# Autodesk Inventor assembly: Aufhängung_Koppeltest
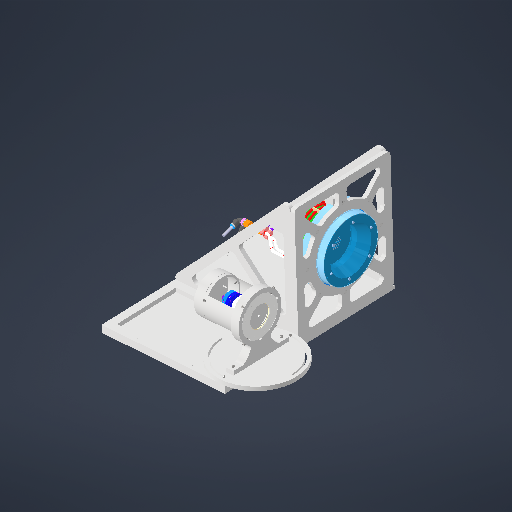
[picture p0: Inventor's stored thumbnail of the model, 512x512]
Saved by Autodesk Inventor 2027 (Build 310192060, 192F)
## iProperties
Created: 2026-07-21
Part Number: Aufhängung_Koppeltest
Document SubType Name: Assembly
Designer: kw
Author: kw
## Documents named in this file (13)
- C:\Users\kw\Documents\ABEP_Koppeltest\Koppeltest_Halterung - Kopie\Aufhängung_Koppeltest.iam
- C:\Users\kw\Documents\ABEP_Koppeltest\Koppeltest_Halterung - Kopie\Aufhängung_Seitenteil.ipt
- C:\Users\kw\Documents\ABEP_Koppeltest\Koppeltest_Halterung - Kopie\Halterung_Teflonplatte.ipt
- C:\Users\kw\Documents\ABEP_Koppeltest\Koppeltest_Halterung - Kopie\Pratze_ISO-K160.ipt
- C:\Users\kw\Documents\ABEP_Koppeltest\19K_001_010_00_A_RIM_10_2019_EFRE_3D_2024_0228\19K_001_010_00_A_RIM_10_2019_EFRE_3D_2024_0228.ipt
- C:\Users\kw\Documents\ABEP_Koppeltest\Koppeltest_Halterung - Kopie\Aufhängung_Front_Koppeltest.ipt
- C:\Users\kw\Documents\ABEP_Koppeltest\Koppeltest_Halterung - Kopie\Aufhängung_Front_RFG_Koppeltest.ipt
- C:\Users\kw\Documents\ABEP_Koppeltest\Koppeltest_Halterung - Kopie\Aufhängung_Drehscheibe.ipt
- C:\Users\kw\Documents\ABEP_Koppeltest\Koppeltest_Halterung - Kopie\Aufhängung_Seitenteil_Koppeltest_außen.ipt
- C:\Users\kw\Documents\ABEP_Koppeltest\RF-Neutralisator\RFN-Setup_Vol3.iam
- C:\Users\kw\OneDrive\Documents\Inventor\Content Center Files\R2027\en-US\ISO 4762(2)\ISO 4762 - M3 x 12ISO.ipt
- C:\Users\kw\OneDrive\Documents\Inventor\Content Center Files\R2027\en-US\ISO 4762(2)\ISO 4762 - M3 x 16ISO.ipt
- C:\Users\kw\OneDrive\Documents\Inventor\Content Center Files\R2027\en-US\ISO 4762(2)\ISO 4762 - M3 x 20ISO.ipt
## Components (18 placed, 12 different names)
1. Aufhängung_Seitenteil:1 — Flush:2, Flush:3, Mate:17, Mate:37, Mate:38
2. Pratze_ISO-K160:4 — Mate:5, Flush:7, Mate:28
3. 19K_001_010_00_A_RIM_10_2019_EFRE_3D_2024_0228:1 — Mate:3, Mate:4, Mate:28
4. Aufhängung_Front_Koppeltest:1 — Mate:2, Flush:5, Mate:3, Mate:4, Mate:5, Flush:7, Flush:13
5. Halterung_Teflonplatte:1 — Flush:2, Flush:3, Mate:2, Flush:5, Mate:17, Flush:13, Mate:37, Mate:38, Mate:39, Flush:17, Flush:18, Mate:40, Flush:19, Mate:41, Mate:42, Mate:43, Mate:44
6. Aufhängung_Front_RFG_Koppeltest:1 — Mate:16, Mate:32, Mate:33, Mate:34, Mate:35, Flush:16, Insert:1, Insert:2
7. Aufhängung_Drehscheibe:1 — Mate:16, Mate:32, Mate:33, Mate:47, Mate:48, Mate:49, Mate:50, Mate:51
8. Aufhängung_Seitenteil_Koppeltest_außen:1 — Mate:40, Flush:19, Mate:41, Mate:42, Mate:43, Mate:44, Mate:47, Mate:52, Mate:53
9. RFN-Setup_Vol3:1 [sub-assembly] — Mate:34, Mate:36, Flush:16
10. Aufhängung_Seitenteil:2 — Mate:39, Flush:17, Flush:18
11. ISO 4762 M3 x 16:1 — Mate:48, Mate:51, Mate:53
12. ISO 4762 M3 x 16:2 — Mate:49, Mate:50, Mate:52
13. ISO 4762 M3 x 20:1 — Insert:1
14. ISO 4762 M3 x 20:2 — Insert:2
15. ISO 4762 M3 x 12:1 — Mate:35, Mate:36
16. ISO 4762 M3 x 12:2
17. ISO 4762 M3 x 12:3
18. ISO 4762 M3 x 12:4
## Component patterns: (4 elements, first: ISO 4762 M3 x 12:1)
## Relationships (38: Mate 27, Flush 9, Insert 2)
- Flush:2: Aufhängung_Seitenteil:1 ↔ Halterung_Teflonplatte:1
- Flush:3 (-10 mm): Aufhängung_Seitenteil:1 ↔ Halterung_Teflonplatte:1
- Mate:2: Aufhängung_Front_Koppeltest:1 ↔ Halterung_Teflonplatte:1
- Flush:5: Aufhängung_Front_Koppeltest:1 ↔ Halterung_Teflonplatte:1
- Mate:3: 19K_001_010_00_A_RIM_10_2019_EFRE_3D_2024_0228:1 ↔ Aufhängung_Front_Koppeltest:1
- Mate:4: 19K_001_010_00_A_RIM_10_2019_EFRE_3D_2024_0228:1 ↔ Aufhängung_Front_Koppeltest:1
- Mate:5: Pratze_ISO-K160:4 ↔ Aufhängung_Front_Koppeltest:1
- Flush:7 (0.5 mm): Pratze_ISO-K160:4 ↔ Aufhängung_Front_Koppeltest:1
- Mate:16: Aufhängung_Front_RFG_Koppeltest:1 ↔ Aufhängung_Drehscheibe:1
- Mate:17: Aufhängung_Seitenteil:1 ↔ Halterung_Teflonplatte:1
- Flush:13: Aufhängung_Front_Koppeltest:1 ↔ Halterung_Teflonplatte:1
- Mate:28: Pratze_ISO-K160:4 ↔ 19K_001_010_00_A_RIM_10_2019_EFRE_3D_2024_0228:1
- Mate:32: Aufhängung_Front_RFG_Koppeltest:1 ↔ Aufhängung_Drehscheibe:1
- Mate:33: Aufhängung_Front_RFG_Koppeltest:1 ↔ Aufhängung_Drehscheibe:1
- Mate:34: Aufhängung_Front_RFG_Koppeltest:1 ↔ RFN-Setup_Vol3:1
- Mate:35: Aufhängung_Front_RFG_Koppeltest:1 ↔ ISO 4762 M3 x 12:1
- Mate:36: RFN-Setup_Vol3:1 ↔ ISO 4762 M3 x 12:1
- Flush:16: Aufhängung_Front_RFG_Koppeltest:1 ↔ RFN-Setup_Vol3:1
- Mate:37: Aufhängung_Seitenteil:1 ↔ Halterung_Teflonplatte:1
- Mate:38: Aufhängung_Seitenteil:1 ↔ Halterung_Teflonplatte:1
- Mate:39: Halterung_Teflonplatte:1 ↔ Aufhängung_Seitenteil:2
- Flush:17 (10 mm): Halterung_Teflonplatte:1 ↔ Aufhängung_Seitenteil:2
- Flush:18 (250 mm): Halterung_Teflonplatte:1 ↔ Aufhängung_Seitenteil:2
- Mate:40: Halterung_Teflonplatte:1 ↔ Aufhängung_Seitenteil_Koppeltest_außen:1
- Flush:19: Halterung_Teflonplatte:1 ↔ Aufhängung_Seitenteil_Koppeltest_außen:1
- Mate:41: Halterung_Teflonplatte:1 ↔ Aufhängung_Seitenteil_Koppeltest_außen:1
- Mate:42: Halterung_Teflonplatte:1 ↔ Aufhängung_Seitenteil_Koppeltest_außen:1
- Mate:43: Halterung_Teflonplatte:1 ↔ Aufhängung_Seitenteil_Koppeltest_außen:1
- Mate:44: Halterung_Teflonplatte:1 ↔ Aufhängung_Seitenteil_Koppeltest_außen:1
- Mate:47: Aufhängung_Drehscheibe:1 ↔ Aufhängung_Seitenteil_Koppeltest_außen:1
- Mate:48: Aufhängung_Drehscheibe:1 ↔ ISO 4762 M3 x 16:1
- Mate:49: Aufhängung_Drehscheibe:1 ↔ ISO 4762 M3 x 16:2
- Mate:50: Aufhängung_Drehscheibe:1 ↔ ISO 4762 M3 x 16:2
- Mate:51: Aufhängung_Drehscheibe:1 ↔ ISO 4762 M3 x 16:1
- Mate:52: Aufhängung_Seitenteil_Koppeltest_außen:1 ↔ ISO 4762 M3 x 16:2
- Mate:53: Aufhängung_Seitenteil_Koppeltest_außen:1 ↔ ISO 4762 M3 x 16:1
- Insert:1: Aufhängung_Front_RFG_Koppeltest:1 ↔ ISO 4762 M3 x 20:1
- Insert:2: Aufhängung_Front_RFG_Koppeltest:1 ↔ ISO 4762 M3 x 20:2
